# Autodesk Inventor assembly: Nanoscopy-on-a-cheap_v6_dual
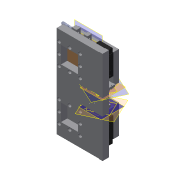
[picture p0: Inventor's stored thumbnail of the model, 180x180]
Saved by Autodesk Inventor 2019 (Build 230136000, 136)
## iProperties
Created: 2019-05-02
Part Number: Nanoscopy-on-a-cheap_v6_dual
Document SubType Name: Assembly
Designer: diederichbenedict
Author: diederichbenedict
## Documents named in this file (11)
- C:\Users\diederichbenedict\Dropbox\Dokumente\Promotion\PROJECTS\STORMoChip\INVENTOR\Nanoscopy-on-a-cheap\Nanoscopy-on-a-cheap_v6_dual.iam
- C:\Users\diederichbenedict\Dropbox\Dokumente\Promotion\PROJECTS\STORMoChip\INVENTOR\Nanoscopy-on-a-cheap\00_ZEISS_Axiotech_Plate.ipt
- C:\Users\diederichbenedict\Dropbox\Dokumente\Promotion\PROJECTS\STORMoChip\INVENTOR\Nanoscopy-on-a-cheap\00_XY_stage-CHUO_SEIKI_LD-647-R1.iam
- C:\Users\diederichbenedict\Dropbox\Dokumente\Promotion\PROJECTS\STORMoChip\INVENTOR\Nanoscopy-on-a-cheap\Assembly_Lasergroup_wPickup_v1.iam
- C:\Users\diederichbenedict\Dropbox\Dokumente\Promotion\PROJECTS\STORMoChip\INVENTOR\Nanoscopy-on-a-cheap\00_Microscope_Objective.ipt
- C:\Users\diederichbenedict\Dropbox\Dokumente\Promotion\PROJECTS\STORMoChip\INVENTOR\Nanoscopy-on-a-cheap\10_Adapter_Laser_XY_left.ipt
- C:\Users\diederichbenedict\Dropbox\Dokumente\Promotion\PROJECTS\STORMoChip\INVENTOR\Nanoscopy-on-a-cheap\02_Nanoscopy_Chip.ipt
- C:\Users\diederichbenedict\Dropbox\Dokumente\Promotion\PROJECTS\STORMoChip\INVENTOR\Nanoscopy-on-a-cheap\10_Baseplate.ipt
- C:\Users\diederichbenedict\Dropbox\Dokumente\Promotion\PROJECTS\STORMoChip\INVENTOR\Nanoscopy-on-a-cheap\10_Baseplate_Axiotech_mono.ipt
- C:\Users\diederichbenedict\Dropbox\Dokumente\Promotion\PROJECTS\STORMoChip\INVENTOR\Nanoscopy-on-a-cheap\00_Metalsheet_1mm_30x40.ipt
- C:\Users\diederichbenedict\Dropbox\Dokumente\Promotion\PROJECTS\STORMoChip\INVENTOR\Nanoscopy-on-a-cheap\10_Adapter_Laser_XY_right.ipt
## Components (13 placed, 10 different names)
1. 00_ZEISS_Axiotech_Plate:1 — Mate:13
2. 00_XY_stage-CHUO_SEIKI_LD-647-R1:1 [sub-assembly] — Flush:11, Flush:12, Flush:22, Flush:23, Flush:24, Flush:25, Flush:26
3. 02_Nanoscopy_Chip:1 — Mate:17
4. 00_Microscope_Objective:1 — Mate:13
5. 10_Adapter_Laser_XY_left:1 — Flush:11, Flush:12, Mate:18, Flush:30, Mate:19
6. 10_Baseplate:1 — Flush:22, Flush:23
7. 10_Baseplate_Axiotech_mono:1 — Flush:24, Flush:25, Flush:26, Angle:3, Mate:20, Insert:21, Angle:4
8. 00_Metalsheet_1mm_30x40:1 — Angle:3, Mate:17
9. Assembly_Lasergroup_wPickup_v1:1 [sub-assembly] — Mate:18, Flush:30, Mate:19, Mate:21, Flush:31, Mate:22
10. 02_Nanoscopy_Chip:2 — Mate:20, Mate:21, Flush:31
11. 00_XY_stage-CHUO_SEIKI_LD-647-R1:2 [sub-assembly] — Insert:21, Angle:4, Insert:22, Angle:5
12. 10_Adapter_Laser_XY_right:1 — Insert:22, Angle:5, Insert:23
13. Assembly_Lasergroup_wPickup_v1:2 [sub-assembly] — Mate:22, Insert:23
## Relationships (24: Flush 9, Mate 7, Insert 4, Angle 4)
- Flush:11: 00_XY_stage-CHUO_SEIKI_LD-647-R1:1 ↔ 10_Adapter_Laser_XY_left:1
- Flush:12: 00_XY_stage-CHUO_SEIKI_LD-647-R1:1 ↔ 10_Adapter_Laser_XY_left:1
- Mate:13 (30 mm): 00_ZEISS_Axiotech_Plate:1 ↔ 00_Microscope_Objective:1
- [Insert] (5 mm): 02_Nanoscopy_Chip:1 ↔ 00_Microscope_Objective:1
- [Angle] (180 deg): 02_Nanoscopy_Chip:1 ↔ 10_Adapter_Laser_XY_left:1
- Flush:22: 00_XY_stage-CHUO_SEIKI_LD-647-R1:1 ↔ 10_Baseplate:1
- Flush:23: 00_XY_stage-CHUO_SEIKI_LD-647-R1:1 ↔ 10_Baseplate:1
- Flush:24: 00_XY_stage-CHUO_SEIKI_LD-647-R1:1 ↔ 10_Baseplate_Axiotech_mono:1
- Flush:25: 00_XY_stage-CHUO_SEIKI_LD-647-R1:1 ↔ 10_Baseplate_Axiotech_mono:1
- Flush:26: 00_XY_stage-CHUO_SEIKI_LD-647-R1:1 ↔ 10_Baseplate_Axiotech_mono:1
- Angle:3 (180 deg): 10_Baseplate_Axiotech_mono:1 ↔ 00_Metalsheet_1mm_30x40:1
- Mate:17: 02_Nanoscopy_Chip:1 ↔ 00_Metalsheet_1mm_30x40:1
- Mate:18: 10_Adapter_Laser_XY_left:1 ↔ Assembly_Lasergroup_wPickup_v1:1
- Flush:30: 10_Adapter_Laser_XY_left:1 ↔ Assembly_Lasergroup_wPickup_v1:1
- Mate:19: 10_Adapter_Laser_XY_left:1 ↔ Assembly_Lasergroup_wPickup_v1:1
- Mate:20 (5 mm): 10_Baseplate_Axiotech_mono:1 ↔ 02_Nanoscopy_Chip:2
- Mate:21 (2 mm): Assembly_Lasergroup_wPickup_v1:1 ↔ 02_Nanoscopy_Chip:2
- Flush:31 (5 mm): Assembly_Lasergroup_wPickup_v1:1 ↔ 02_Nanoscopy_Chip:2
- Insert:21: 10_Baseplate_Axiotech_mono:1 ↔ 00_XY_stage-CHUO_SEIKI_LD-647-R1:2
- Angle:4 (180 deg): 10_Baseplate_Axiotech_mono:1 ↔ 00_XY_stage-CHUO_SEIKI_LD-647-R1:2
- Insert:22: 00_XY_stage-CHUO_SEIKI_LD-647-R1:2 ↔ 10_Adapter_Laser_XY_right:1
- Angle:5 (180 deg): 00_XY_stage-CHUO_SEIKI_LD-647-R1:2 ↔ 10_Adapter_Laser_XY_right:1
- Mate:22: Assembly_Lasergroup_wPickup_v1:1 ↔ Assembly_Lasergroup_wPickup_v1:2
- Insert:23: 10_Adapter_Laser_XY_right:1 ↔ Assembly_Lasergroup_wPickup_v1:2
